# Autodesk Inventor assembly: Mock Module PCB
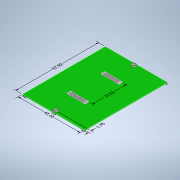
[picture p0: Inventor's stored thumbnail of the model, 180x180]
Saved by Autodesk Inventor 2022 (Build 260153000, 153)
## iProperties
Created: 2021-07-19
Part Number: Mock Module PCB
Document SubType Name: Assembly
Designer: Caleb
Author: Caleb
## Documents named in this file (5)
- C:\Users\Caleb\Desktop\nebraska-silicon-lab\Hardware\ETL\modules\tamale v1.4\Mock Module PCB - v1p4.iam
- C:\Users\Caleb\Desktop\nebraska-silicon-lab\Hardware\ETL\ETL-SH-Design\3D-model\K3D-WP7B-S050VA1-V3_JAE_Proprietary v1_14.iam
- C:\Users\Caleb\Desktop\nebraska-silicon-lab\Hardware\ETL\modules\tamale v1.4\Mock Module PCB - v1p4.ipt
- C:\Users\Caleb\Desktop\nebraska-silicon-lab\Hardware\ETL\modules\tamale v1.4\inter-board spacer - v1.ipt
- C:\Users\Caleb\Desktop\nebraska-silicon-lab\Hardware\ETL\modules\tamale v1.4\underboard spacer - v1.ipt
## Components (11 placed, 4 different names)
1. Mock Module PCB - v1p4:1 — Mate:1, Mate:2, Flush:4, Flush:6, Insert:1, Insert:2, Mate:3, Angle:1, Flush:7, Mate:4, Flush:8, Flush:9, Mate:5, Mate:6, Flush:11, Flush:12, Flush:13, Flush:14, Mate:7, Flush:15, Flush:16, Flush:17, Mate:8, Flush:18
2. K3D-WP7B-S050VA1-V3_JAE_Proprietary v1_14:1 [sub-assembly] — Mate:1, Flush:3, Flush:5
3. K3D-WP7B-S050VA1-V3_JAE_Proprietary v1_14:2 [sub-assembly] — Mate:2, Flush:3, Flush:4, Flush:5, Flush:6
4. inter-board spacer - v1:1 — Insert:1
5. inter-board spacer - v1:2 — Insert:2
6. underboard spacer - v1:1 — Mate:3, Angle:1, Flush:7, Flush:10
7. underboard spacer - v1:2 — Mate:4, Flush:8, Flush:9, Flush:10
8. underboard spacer - v1:3 — Mate:6, Flush:11, Flush:12
9. underboard spacer - v1:4 — Mate:5, Flush:13, Flush:14
10. underboard spacer - v1:5 — Mate:7, Flush:15, Flush:16
11. underboard spacer - v1:6 — Flush:17, Mate:8, Flush:18
## Relationships (27: Flush 16, Mate 8, Insert 2, Angle 1)
- Mate:1: Mock Module PCB - v1p4:1 ↔ K3D-WP7B-S050VA1-V3_JAE_Proprietary v1_14:1
- Mate:2: Mock Module PCB - v1p4:1 ↔ K3D-WP7B-S050VA1-V3_JAE_Proprietary v1_14:2
- Flush:3 (23.531 mm): K3D-WP7B-S050VA1-V3_JAE_Proprietary v1_14:1 ↔ K3D-WP7B-S050VA1-V3_JAE_Proprietary v1_14:2
- Flush:4 (15.7945 mm): Mock Module PCB - v1p4:1 ↔ K3D-WP7B-S050VA1-V3_JAE_Proprietary v1_14:2
- Flush:5: K3D-WP7B-S050VA1-V3_JAE_Proprietary v1_14:1 ↔ K3D-WP7B-S050VA1-V3_JAE_Proprietary v1_14:2
- Flush:6 (15.307 mm): Mock Module PCB - v1p4:1 ↔ K3D-WP7B-S050VA1-V3_JAE_Proprietary v1_14:2
- Insert:1: Mock Module PCB - v1p4:1 ↔ inter-board spacer - v1:1
- Insert:2: Mock Module PCB - v1p4:1 ↔ inter-board spacer - v1:2
- Mate:3: Mock Module PCB - v1p4:1 ↔ underboard spacer - v1:1
- Angle:1 (0 deg): Mock Module PCB - v1p4:1 ↔ underboard spacer - v1:1
- Flush:7: Mock Module PCB - v1p4:1 ↔ underboard spacer - v1:1
- Mate:4: Mock Module PCB - v1p4:1 ↔ underboard spacer - v1:2
- Flush:8: Mock Module PCB - v1p4:1 ↔ underboard spacer - v1:2
- Flush:9 (20.45 mm): Mock Module PCB - v1p4:1 ↔ underboard spacer - v1:2
- Flush:10: underboard spacer - v1:1 ↔ underboard spacer - v1:2
- Mate:5: Mock Module PCB - v1p4:1 ↔ underboard spacer - v1:4
- Mate:6: Mock Module PCB - v1p4:1 ↔ underboard spacer - v1:3
- Flush:11: Mock Module PCB - v1p4:1 ↔ underboard spacer - v1:3
- Flush:12: Mock Module PCB - v1p4:1 ↔ underboard spacer - v1:3
- Flush:13: Mock Module PCB - v1p4:1 ↔ underboard spacer - v1:4
- Flush:14: Mock Module PCB - v1p4:1 ↔ underboard spacer - v1:4
- Mate:7: Mock Module PCB - v1p4:1 ↔ underboard spacer - v1:5
- Flush:15: Mock Module PCB - v1p4:1 ↔ underboard spacer - v1:5
- Flush:16: Mock Module PCB - v1p4:1 ↔ underboard spacer - v1:5
- Flush:17: Mock Module PCB - v1p4:1 ↔ underboard spacer - v1:6
- Mate:8: Mock Module PCB - v1p4:1 ↔ underboard spacer - v1:6
- Flush:18: Mock Module PCB - v1p4:1 ↔ underboard spacer - v1:6
